# Autodesk Inventor assembly: cam roller assembly
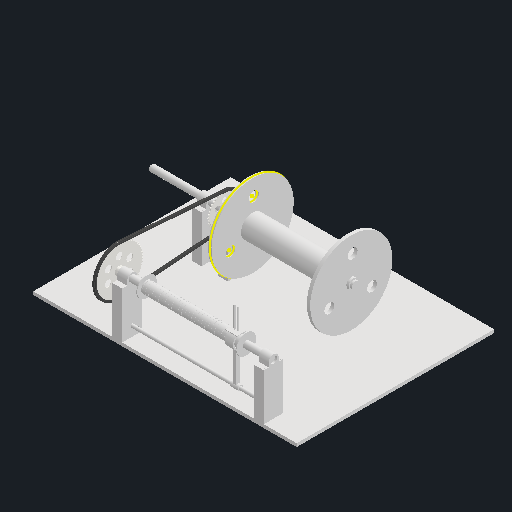
[picture p0: Inventor's stored thumbnail of the model, 512x512]
Saved by Autodesk Inventor 2026.1 (Build 301233020, 233B)
## iProperties
Created: 2025-12-30
Part Number: cam roller assembly
Document SubType Name: Assembly
Designer: Austin Ngobeni
Author: Austin Ngobeni
## Documents named in this file (7)
- C:\Users\kngob\projects\Inventor\cam-roller\cam roller assembly.iam
- C:\Users\kngob\projects\Inventor\cam-roller\parts\base.ipt
- C:\Users\kngob\projects\Inventor\cam-roller\cam roller assembly\Design Accelerator\Chain Drive1.iam
- C:\Users\kngob\projects\Inventor\cam-roller\parts\hold down pin.ipt
- C:\Users\kngob\projects\Inventor\cam-roller\parts\roller.ipt
- C:\Users\kngob\projects\Inventor\cam-roller\parts\cam shaft.ipt
- C:\Users\kngob\projects\Inventor\cam-roller\parts\guide.ipt
## Components (9 placed, 6 different names)
1. base:1 — Flush:1, Flush:2, Flush:3, Flush:4, Flush:5, Flush:6, Flush:7, Mate:3, Flush:8, Flush:9, Mate:4, Mate:10, Flush:10, Flush:11, Mate:11
2. Chain Drive:1 [sub-assembly] — Mate:5
3. hold down pin:1 — Flush:6, Flush:7, Mate:4, Mate:5
4. hold down pin:2 — Flush:4, Flush:5
5. hold down pin:3 — Mate:3, Flush:8, Flush:9, Mate:6, Mate:7
6. roller:1 — Mate:6, Mate:7
7. cam shaft:1
8. hold down pin:4 — Mate:10, Flush:10, Flush:11
9. guide:1 — Mate:11
## Relationships (18: Flush 11, Mate 7)
- Flush:1: base:1
- Flush:2: base:1
- Flush:3: base:1
- Flush:4: base:1 ↔ hold down pin:2
- Flush:5: base:1 ↔ hold down pin:2
- Flush:6: base:1 ↔ hold down pin:1
- Flush:7: base:1 ↔ hold down pin:1
- Mate:3: base:1 ↔ hold down pin:3
- Flush:8: base:1 ↔ hold down pin:3
- Flush:9: base:1 ↔ hold down pin:3
- Mate:4: base:1 ↔ hold down pin:1
- Mate:5: Chain Drive:1 ↔ hold down pin:1
- Mate:6: hold down pin:3 ↔ roller:1
- Mate:7: hold down pin:3 ↔ roller:1
- Mate:10: base:1 ↔ hold down pin:4
- Flush:10: base:1 ↔ hold down pin:4
- Flush:11: base:1 ↔ hold down pin:4
- Mate:11: base:1 ↔ guide:1
